# Autodesk Inventor assembly: KSTI-16
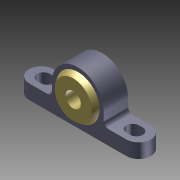
[picture p0: Inventor's stored thumbnail of the model, 180x180]
Saved by Autodesk Inventor 2011 (Build 150239000, 239)
## iProperties
Category: Plastic Bearings
Created: 2007-11-11
Part Number: KSTI-16
Document SubType Name: Assembly
Designer: Brent
Catalog Web Link: http://www.igus.com/igcat/ig_cat1.asp?p=ig_26_2.gif
Description: igubal Pillow Block Bearing
Vendor: igus
Mass: 99.8703 g
Surface Area: 269.768 cm^2
Volume: 83.6297 cm^3
Density: 1.1942 g/cm^3
Project: FIRST
Title: igubal Pillow Block Bearing
Author: Autodesk, Inc.
## Documents named in this file (3)
- R:\2012\Inventor\vkop\Plastic-Bearings\Plastic Bearings_igus_KSTI-16.iam
- R:\2012\Inventor\vkop\Plastic-Bearings\KSTI-16_Housing.ipt
- R:\2012\Inventor\vkop\Plastic-Bearings\KSTI-16_Spherical Bearing.ipt
## Components (2 placed, 2 different names)
1. KSTI-16_Housing:1 — Mate:1, Angle:1
2. KSTI-16_Spherical Bearing:1 — Mate:1, Angle:1
## Relationships (2: Mate 1, Angle 1)
- Mate:1: KSTI-16_Housing:1 ↔ KSTI-16_Spherical Bearing:1
- Angle:1 (0 deg): KSTI-16_Housing:1 ↔ KSTI-16_Spherical Bearing:1
